# Autodesk Inventor assembly: Anpresspinns_Assembly
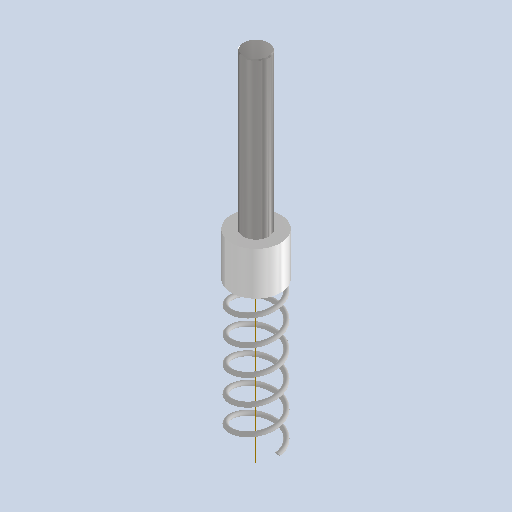
[picture p0: Inventor's stored thumbnail of the model, 512x512]
Saved by Autodesk Inventor 2024 (Build 280153000, 153)
## iProperties
Created: 2022-08-21
Part Number: Anpresspinns_Assembly
Document SubType Name: Assembly
Designer: alexw
Mass: 1.40869 g
Surface Area: 5.46921 cm^2
Volume: 0.285717 cm^3
Density: 4.93039 g/cm^3
Author: alexw
## Documents named in this file (4)
- C:\Users\AEWALDER\Documents\Inventor\03_CurrentProjects\MasterThesis\PSM_V1_Rillenkugellager\Ueberarbeiteter DaVincikopf\Anpresspinns_Assembly.iam
- C:\Users\AEWALDER\Documents\Inventor\03_CurrentProjects\MasterThesis\PSM_V1_Rillenkugellager\Ueberarbeiteter DaVincikopf\AnpresspinnAufnahme_Buchse.ipt
- C:\Users\AEWALDER\Documents\Inventor\03_CurrentProjects\MasterThesis\PSM_V1_Rillenkugellager\Ueberarbeiteter DaVincikopf\Anpresspinns.ipt
- C:\Users\AEWALDER\Documents\Inventor\03_CurrentProjects\MasterThesis\PSM_V1_Rillenkugellager\Maschinenbauteil\rdf-1369-0.ipt
## Components (3 placed, 3 different names)
1. AnpresspinnAufnahme_Buchse:1 — Passend:1, Passend:2, Passend:3, Passend:4, Passend:5, Passend:6, Passend:7
2. Anpresspinns:1 — Passend:4, Passend:5
3. rdf-1369-0:1 — Passend:6, Passend:7
## Relationships (7: Mate 7)
- Passend:1 [Mate]: AnpresspinnAufnahme_Buchse:1
- Passend:2 [Mate]: AnpresspinnAufnahme_Buchse:1
- Passend:3 [Mate]: AnpresspinnAufnahme_Buchse:1
- Passend:4 [Mate]: AnpresspinnAufnahme_Buchse:1 ↔ Anpresspinns:1
- Passend:5 [Mate]: AnpresspinnAufnahme_Buchse:1 ↔ Anpresspinns:1
- Passend:6 [Mate]: AnpresspinnAufnahme_Buchse:1 ↔ rdf-1369-0:1
- Passend:7 [Mate]: AnpresspinnAufnahme_Buchse:1 ↔ rdf-1369-0:1
